# Autodesk Inventor assembly: SuperBlock US
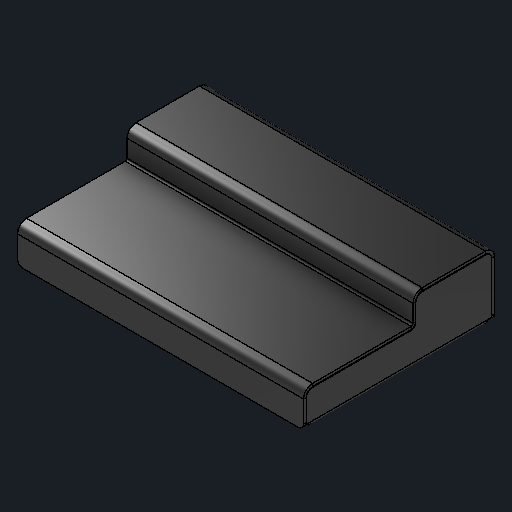
[picture p0: Inventor's stored thumbnail of the model, 512x512]
Saved by Autodesk Inventor 2026.2 (Build 302298000, 298)
## iProperties
Created: 2026-06-19
Part Number: SuperBlock US
Document SubType Name: Assembly
Designer: JoshuaEah
Author: JoshuaEah
## Documents named in this file (3)
- C:\Users\JoshuaEah\Documents\GitHub\Designed-Trinkets\Guitar\Modular Pedalboard\Pedals\SuperBlock US\SuperBlock US.iam
- C:\Users\JoshuaEah\Documents\GitHub\Designed-Trinkets\Guitar\Modular Pedalboard\Pedals\SuperBlock US\Top Shell.ipt
- C:\Users\JoshuaEah\Documents\GitHub\Designed-Trinkets\Guitar\Modular Pedalboard\Pedals\SuperBlock US\Bottom Shell.ipt
## Components (2 placed, 2 different names)
1. Top Shell:1 — Mate:1, Flush:1, Mate:2
2. Bottom Shell:1 — Mate:1, Flush:1, Mate:2
## Relationships (3: Mate 2, Flush 1)
- Mate:1: Top Shell:1 ↔ Bottom Shell:1
- Flush:1: Top Shell:1 ↔ Bottom Shell:1
- Mate:2 (0.4 mm): Top Shell:1 ↔ Bottom Shell:1
